# Autodesk Inventor assembly: main
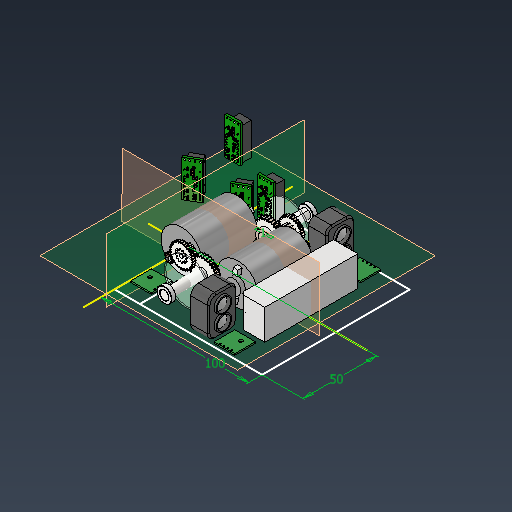
[picture p0: Inventor's stored thumbnail of the model, 512x512]
Saved by Autodesk Inventor 2026.2 (Build 302298010, 298A)
## iProperties
Created: 2026-03-09
Part Number: main
Document SubType Name: Assembly
Designer: szymo
Author: szymo
## Documents named in this file (6)
- D:\tech\robotyka\robots\evangelion-turbo\inventor-project\main.iam
- D:\tech\robotyka\robots\evangelion-turbo\inventor-project\drive-train.iam
- D:\tech\robotyka\robots\evangelion-turbo\inventor-project\LUNA.ipt
- D:\tech\robotyka\robots\evangelion-turbo\inventor-project\3s450mah.ipt
- D:\tech\robotyka\robots\evangelion-turbo\inventor-project\sharp\sharp\sharp.ipt
- D:\tech\robotyka\robots\evangelion-turbo\inventor-project\KTIR-Board.ipt
## Components (12 placed, 5 different names)
1. drive-train:1 [sub-assembly] — Flush:2, Flush:3, Flush:4, Mate:2, Mate:3, Tangent:1
2. 3s450mah:1 — Flush:8, Tangent:1, Flush:9
3. KTIR-Board:5
4. sharp:6
5. sharp:7
6. sharp:5 — Mate:10, Flush:22, Mate:11, Mate:13
7. sharp:4 — Flush:23, Angle:3, Mate:12, Mate:13
8. KTIR-Board:4 — Flush:17, Flush:19, Flush:21
9. LUNA:2 — Mate:1, Mate:3, Angle:2, Flush:7
10. LUNA:1 — Flush:5, Mate:2, Angle:1, Flush:6
11. KTIR-Board:1 — Flush:10, Flush:11, Flush:13
12. KTIR-Board:2 — Mate:4, Flush:12, Flush:14
## Relationships (31: Flush 19, Mate 8, Angle 3, Tangent 1)
- Flush:1 (-101.75 mm)
- Flush:2: drive-train:1
- Flush:3 (-18.4 mm): drive-train:1
- Flush:4: drive-train:1
- Flush:5 (49.5 mm): LUNA:1
- Mate:1 (-49.5 mm): LUNA:2
- Mate:2 (18 mm): drive-train:1 ↔ LUNA:1
- Mate:3 (18 mm): drive-train:1 ↔ LUNA:2
- Angle:1 (0 deg): LUNA:1
- Angle:2 (180 deg): LUNA:2
- Flush:6: LUNA:1
- Flush:7: LUNA:2
- Flush:8 (1 mm): 3s450mah:1
- Tangent:1: drive-train:1 ↔ 3s450mah:1
- Flush:9 (-31 mm): 3s450mah:1
- Flush:10 (-49.5 mm): KTIR-Board:1
- Mate:4 (-49.5 mm): KTIR-Board:2
- Flush:11 (0.13 mm): KTIR-Board:1
- Flush:12 (0.13 mm): KTIR-Board:2
- Flush:13 (67 mm): KTIR-Board:1
- Flush:14 (-67 mm): KTIR-Board:2
- Flush:17 (-1 mm): KTIR-Board:4
- Flush:19 (2 mm): KTIR-Board:4
- Flush:21 (-23.5 mm): KTIR-Board:4
- Mate:10 (-16.681 mm): sharp:5
- Flush:22 (0.5 mm): sharp:5
- Mate:11 (-49.5 mm): sharp:5
- Flush:23 (2 mm): sharp:4
- Angle:3 (60 deg): sharp:4
- Mate:12 (-0.5 mm): sharp:4
- Mate:13 (1 mm): sharp:5 ↔ sharp:4
